# Autodesk Inventor assembly: EnsambleAislante
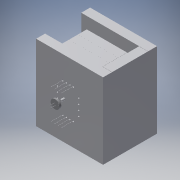
[picture p0: Inventor's stored thumbnail of the model, 180x180]
Saved by Autodesk Inventor 2017 (Build 210142000, 142)
## iProperties
Created: 2021-02-12
Part Number: EnsambleAislante
Document SubType Name: Assembly
Designer: USUARIO
Author: USUARIO
## Documents named in this file (8)
- D:\Laboratorio\Mufla\2021\Mufla 3L Psoc Artilab #0045886XX OP2021128\Modelo\EnsambleAislante.iam
- D:\Laboratorio\Mufla\2021\Mufla 3L Psoc Artilab #0045886XX OP2021128\Modelo\TapaFrontal.ipt
- D:\Laboratorio\Mufla\2021\Mufla 3L Psoc Artilab #0045886XX OP2021128\Modelo\PiezaInferior.ipt
- D:\Laboratorio\Mufla\2021\Mufla 3L Psoc Artilab #0045886XX OP2021128\Modelo\Piso.ipt
- D:\Laboratorio\Mufla\2021\Mufla 3L Psoc Artilab #0045886XX OP2021128\Modelo\Lateral.ipt
- D:\Laboratorio\Mufla\2021\Mufla 3L Psoc Artilab #0045886XX OP2021128\Modelo\Trasera.ipt
- D:\Laboratorio\Mufla\2021\Mufla 3L Psoc Artilab #0045886XX OP2021128\Modelo\Resistencia3.ipt
- D:\Laboratorio\Mufla\2021\Mufla 3L Psoc Artilab #0045886XX OP2021128\Modelo\Termocupla\Termocupla.iam
## Components (24 placed, 7 different names)
1. TapaFrontal:1 — Flush:44, Flush:45, Flush:46, Flush:47, Mate:39, Flush:82, Flush:83, Mate:63
2. PiezaInferior:1 — Flush:46, Flush:47, Mate:39, Mate:40, Flush:48, Flush:49, Mate:41, Flush:50
3. Piso:1 — Flush:44, Flush:45, Mate:63, Mate:64
4. PiezaInferior:5 — Mate:43, Flush:51, Mate:44, Mate:50, Flush:56
5. Lateral:1 — Mate:40, Flush:48, Flush:49, Mate:42, Mate:43, Flush:51, Mate:44, Flush:57
6. Lateral:5 — Mate:41, Flush:50, Mate:42
7. Trasera:1 — Flush:82, Flush:83, Mate:64, Insert:1
8. PiezaInferior:6
9. PiezaInferior:7 — Mate:50, Flush:56, Mate:56, Flush:62
10. Lateral:6 — Flush:57, Flush:63
11. Lateral:7
12. PiezaInferior:8
13. PiezaInferior:9 — Mate:56, Flush:62, Mate:62, Flush:68
14. Lateral:8 — Flush:63, Flush:69
15. Lateral:9
16. PiezaInferior:10
17. PiezaInferior:11 — Mate:62, Flush:68
18. Lateral:10 — Flush:69
19. Lateral:11
20. Resistencia3:2
21. Resistencia3:3
22. Resistencia3:4
23. Resistencia3:5
24. Termocupla:1 [sub-assembly] — Insert:1
## Relationships (55: Flush 28, Mate 26, Insert 1)
- Flush:44: TapaFrontal:1 ↔ Piso:1
- Flush:45: TapaFrontal:1 ↔ Piso:1
- Flush:46: TapaFrontal:1 ↔ PiezaInferior:1
- Flush:47 (64.1 mm): TapaFrontal:1 ↔ PiezaInferior:1
- Mate:39: TapaFrontal:1 ↔ PiezaInferior:1
- Mate:40: PiezaInferior:1 ↔ Lateral:1
- Flush:48: PiezaInferior:1 ↔ Lateral:1
- Flush:49: PiezaInferior:1 ↔ Lateral:1
- Mate:41: PiezaInferior:1 ↔ Lateral:5
- Flush:50: PiezaInferior:1 ↔ Lateral:5
- Mate:42 (-300.483 mm): Lateral:1 ↔ Lateral:5
- Mate:43: PiezaInferior:5 ↔ Lateral:1
- Flush:51: PiezaInferior:5 ↔ Lateral:1
- Mate:44: PiezaInferior:5 ↔ Lateral:1
- [Mate]: PiezaInferior:6 ↔ Lateral:6
- [Flush]: PiezaInferior:6 ↔ Lateral:6
- [Flush]: PiezaInferior:6 ↔ Lateral:6
- [Mate]: PiezaInferior:6 ↔ Lateral:7
- [Flush]: PiezaInferior:6 ↔ Lateral:7
- [Mate] (-300.483 mm): Lateral:6 ↔ Lateral:7
- [Mate]: PiezaInferior:7 ↔ Lateral:6
- [Flush]: PiezaInferior:7 ↔ Lateral:6
- [Mate]: PiezaInferior:7 ↔ Lateral:6
- Mate:50: PiezaInferior:5 ↔ PiezaInferior:7
- Flush:56: PiezaInferior:5 ↔ PiezaInferior:7
- Flush:57: Lateral:1 ↔ Lateral:6
- [Mate]: PiezaInferior:8 ↔ Lateral:8
- [Flush]: PiezaInferior:8 ↔ Lateral:8
- [Flush]: PiezaInferior:8 ↔ Lateral:8
- [Mate]: PiezaInferior:8 ↔ Lateral:9
- [Flush]: PiezaInferior:8 ↔ Lateral:9
- [Mate] (-300.483 mm): Lateral:8 ↔ Lateral:9
- [Mate]: PiezaInferior:9 ↔ Lateral:8
- [Flush]: PiezaInferior:9 ↔ Lateral:8
- [Mate]: PiezaInferior:9 ↔ Lateral:8
- Mate:56: PiezaInferior:7 ↔ PiezaInferior:9
- Flush:62: PiezaInferior:7 ↔ PiezaInferior:9
- Flush:63: Lateral:6 ↔ Lateral:8
- [Mate]: PiezaInferior:10 ↔ Lateral:10
- [Flush]: PiezaInferior:10 ↔ Lateral:10
- [Flush]: PiezaInferior:10 ↔ Lateral:10
- [Mate]: PiezaInferior:10 ↔ Lateral:11
- [Flush]: PiezaInferior:10 ↔ Lateral:11
- [Mate] (-300.483 mm): Lateral:10 ↔ Lateral:11
- [Mate]: PiezaInferior:11 ↔ Lateral:10
- [Flush]: PiezaInferior:11 ↔ Lateral:10
- [Mate]: PiezaInferior:11 ↔ Lateral:10
- Mate:62: PiezaInferior:9 ↔ PiezaInferior:11
- Flush:68: PiezaInferior:9 ↔ PiezaInferior:11
- Flush:69: Lateral:8 ↔ Lateral:10
- Flush:82: TapaFrontal:1 ↔ Trasera:1
- Flush:83: TapaFrontal:1 ↔ Trasera:1
- Mate:63 (1 mm): TapaFrontal:1 ↔ Piso:1
- Mate:64 (1 mm): Piso:1 ↔ Trasera:1
- Insert:1 (-20 mm): Trasera:1 ↔ Termocupla:1
## Named parameters: d139_d132 = -300.483 mm, d140_d136 = 0 mm, d141_d137 = 0 mm, d142_d138 = 0 mm, d143_d127 = 0 mm, d144_d128 = 0 mm, d145_d129 = 0 mm, d146_d130 = 0 mm, d147_d131 = 0 mm, d151_d132 = -300.483 mm, d152_d136 = 0 mm, d153_d137 = 0 mm, d154_d138 = 0 mm, d155_d127 = 0 mm, d156_d128 = 0 mm, d157_d129 = 0 mm, d158_d130 = 0 mm, d159_d131 = 0 mm, d163_d132 = -300.483 mm, d164_d136 = 0 mm, d165_d137 = 0 mm, d166_d138 = 0 mm, d167_d127 = 0 mm, d168_d128 = 0 mm, d169_d129 = 0 mm, d170_d130 = 0 mm, d171_d131 = 0 mm
